# Autodesk Inventor assembly: 1.625 Flex Wheel with Insert
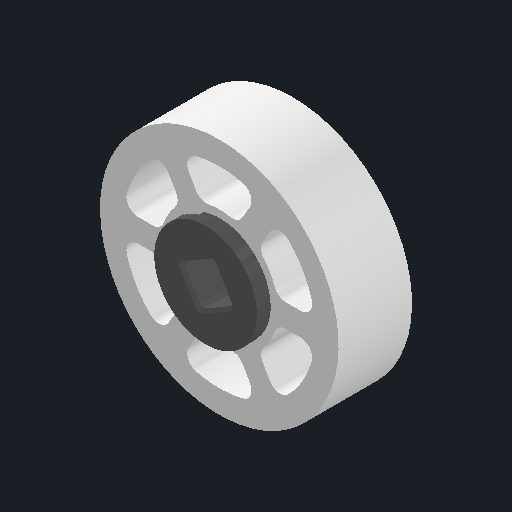
[picture p0: Inventor's stored thumbnail of the model, 512x512]
Saved by Autodesk Inventor 2025.1 (Build 291241020, 241B)
## iProperties
Created: 2024-10-27
Part Number: 1.625 Flex Wheel with Insert
Document SubType Name: Assembly
Designer: Juan
Author: Juan
## Documents named in this file (4)
- C:\Users\Ryan\Documents\GitHub\ATUM-V5RC-High-Stakes-CAD\Robot\Subassemblies\1.625 Flex Wheel with Insert.iam
- C:\Users\Ryan\Documents\GitHub\ATUM-V5RC-High-Stakes-CAD\VEX-CAD-Inventor\Motion\Wheels\Flex Wheels\1.625 Flex Wheel\1.625 30A .500.ipt
- C:\Users\Juan\Documents\GitHub\ATUM-VRC-High-Stakes-CAD\VEX-CAD-Inventor\Motion\Wheels\Flex Wheels\1.625 Flex Wheel.ipt
- C:\Users\Ryan\Documents\GitHub\ATUM-V5RC-High-Stakes-CAD\VEX-CAD-Inventor\Motion\Wheels\Flex Wheels\VersaHex Adapters .250.ipt
## Components (3 placed, 2 different names)
1. 1.625 30A .500:1 — Mate:1, Mate:2, Mate:3, Mate:4, Mate:5
2. VersaHex Adapters .250:1 — Mate:1, Mate:2, Flush:1
3. VersaHex Adapters .250:2 — Mate:3, Mate:4, Flush:1, Mate:5
## Relationships (6: Mate 5, Flush 1)
- Mate:1: 1.625 30A .500:1 ↔ VersaHex Adapters .250:1
- Mate:2: 1.625 30A .500:1 ↔ VersaHex Adapters .250:1
- Mate:3: 1.625 30A .500:1 ↔ VersaHex Adapters .250:2
- Mate:4: 1.625 30A .500:1 ↔ VersaHex Adapters .250:2
- Flush:1: VersaHex Adapters .250:1 ↔ VersaHex Adapters .250:2
- Mate:5: 1.625 30A .500:1 ↔ VersaHex Adapters .250:2
